# Autodesk Inventor assembly: TestAssembly_02
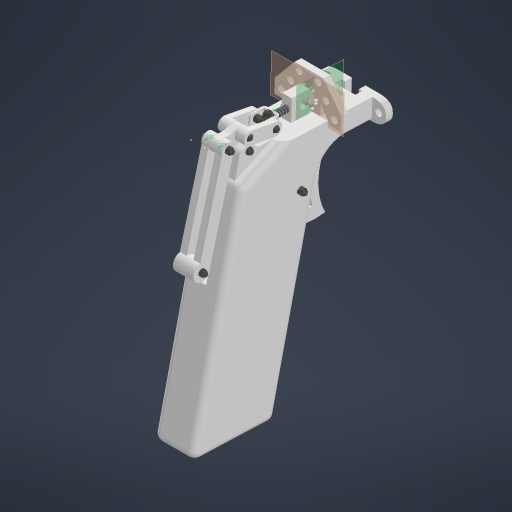
[picture p0: Inventor's stored thumbnail of the model, 512x512]
Saved by Autodesk Inventor 2024.1 (Build 281209000, 209)
## iProperties
Created: 2023-08-23
Part Number: TestAssembly_02
Document SubType Name: Assembly
Designer: Eleanor
Author: Eleanor
## Documents named in this file (13)
- C:\Users\Eleanor\Documents\Inventor\4.5mm ERS\TestAssembly_02.iam
- GripAssembly MK.001.iam
- C:\Users\Eleanor\Documents\Inventor\4.5mm ERS\Trigger.ipt
- C:\Users\Eleanor\Documents\Inventor\4.5mm ERS\TestAssembly_02\Design Accelerator\Clevis Pin Connection1.iam
- C:\Users\Eleanor\Documents\Inventor\4.5mm ERS\UpperLever.ipt
- C:\Users\Eleanor\Documents\Inventor\4.5mm ERS\LowerArm.ipt
- C:\Users\Eleanor\Documents\Inventor\4.5mm ERS\WireBarrelComponent_B.iam
- C:\Users\Eleanor\Documents\Inventor\Content Center Files\R2024\en-US\ISO 7380-1\ISO 7380-1 - M3 x 12.ipt
- C:\Users\Eleanor\Documents\Inventor\4.5mm ERS\FiringPinConnectorPlate.ipt
- C:\Users\Eleanor\Documents\Inventor\4.5mm ERS\FiringPinHolder.ipt
- C:\Users\Eleanor\Documents\Inventor\4.5mm ERS\Compress Spring12.ipt
- C:\Users\Eleanor\Documents\Inventor\4.5mm ERS\TestAssembly_02\Design Accelerator\Clevis Pin Connection2.iam
- C:\Users\Eleanor\Documents\Inventor\4.5mm ERS\Handgrip.iam
## Components (17 placed, 10 different names)
1. Trigger:1 — Mate:6, Mate:12, Mate:14, Mate:31, Mate:58, Mate:59, Mate:60
2. Clevis Pin Connection:1 [sub-assembly] — Mate:5, Mate:6, Mate:52, Mate:59, Mate:62
3. UpperLever:1 — Mate:13, Mate:15, Mate:19, Mate:21, Mate:54, Mate:61
4. LowerArm:1 — Mate:12, Mate:13, Mate:32, Mate:34, Mate:35, Mate:46, Mate:49
5. LowerArm:2 — Mate:14, Mate:15, Mate:57
6. WireBarrelComponent_B:1 [sub-assembly] — Mate:25, Mate:55, Mate:56
7. ISO 7380-1 M3 x 12:1 — Mate:25, Mate:26, Mate:29, Mate:30
8. FiringPinConnectorPlate:1 — Mate:19, Mate:20, Mate:23, Mate:28, Mate:37, Mate:38, Mate:40, Mate:44, Mate:50
9. FiringPinConnectorPlate:2 — Mate:21, Mate:28
10. FiringPinHolder:1 — Mate:20, Mate:23, Mate:26, Mate:29, Flush:2
11. Compress Spring1:1 — Mate:30, Flush:2
12. Clevis Pin Connection:2 [sub-assembly] — Mate:46, Mate:47, Mate:57
13. Clevis Pin Connection:3 [sub-assembly] — Mate:48, Mate:53, Mate:61
14. Clevis Pin Connection:4 [sub-assembly] — Mate:49
15. Clevis Pin Connection:5 [sub-assembly] — Mate:50
16. Clevis Pin Connection:6 [sub-assembly] — Mate:51
17. Handgrip:1 [sub-assembly] — Mate:52, Mate:53, Mate:54, Mate:55, Mate:56, Mate:58, Mate:60, Mate:62
## Relationships (47: Mate 46, Flush 1)
- Mate:3
- Mate:5: Clevis Pin Connection:1
- Mate:6: Trigger:1 ↔ Clevis Pin Connection:1
- Mate:12: Trigger:1 ↔ LowerArm:1
- Mate:13: UpperLever:1 ↔ LowerArm:1
- Mate:14: Trigger:1 ↔ LowerArm:2
- Mate:15: UpperLever:1 ↔ LowerArm:2
- Mate:19: UpperLever:1 ↔ FiringPinConnectorPlate:1
- Mate:20: FiringPinConnectorPlate:1 ↔ FiringPinHolder:1
- Mate:21: UpperLever:1 ↔ FiringPinConnectorPlate:2
- Mate:23: FiringPinConnectorPlate:1 ↔ FiringPinHolder:1
- Mate:25: WireBarrelComponent_B:1 ↔ ISO 7380-1 M3 x 12:1
- Mate:26: ISO 7380-1 M3 x 12:1 ↔ FiringPinHolder:1
- Mate:28: FiringPinConnectorPlate:1 ↔ FiringPinConnectorPlate:2
- Mate:29: ISO 7380-1 M3 x 12:1 ↔ FiringPinHolder:1
- Mate:30: ISO 7380-1 M3 x 12:1 ↔ Compress Spring1:1
- Flush:2: FiringPinHolder:1 ↔ Compress Spring1:1
- Mate:31: Trigger:1
- Mate:32: LowerArm:1
- Mate:33
- Mate:34: LowerArm:1
- Mate:35: LowerArm:1
- Mate:36
- Mate:37: FiringPinConnectorPlate:1
- Mate:38: FiringPinConnectorPlate:1
- Mate:39
- Mate:40: FiringPinConnectorPlate:1
- Mate:43
- Mate:44: FiringPinConnectorPlate:1
- Mate:45
- Mate:46: LowerArm:1 ↔ Clevis Pin Connection:2
- Mate:47: Clevis Pin Connection:2
- Mate:48: Clevis Pin Connection:3
- Mate:49: LowerArm:1 ↔ Clevis Pin Connection:4
- Mate:50: FiringPinConnectorPlate:1 ↔ Clevis Pin Connection:5
- Mate:51: Clevis Pin Connection:6
- Mate:52: Clevis Pin Connection:1 ↔ Handgrip:1
- Mate:53: Clevis Pin Connection:3 ↔ Handgrip:1
- Mate:54: UpperLever:1 ↔ Handgrip:1
- Mate:55: WireBarrelComponent_B:1 ↔ Handgrip:1
- Mate:56: WireBarrelComponent_B:1 ↔ Handgrip:1
- Mate:57: LowerArm:2 ↔ Clevis Pin Connection:2
- Mate:58: Trigger:1 ↔ Handgrip:1
- Mate:59: Trigger:1 ↔ Clevis Pin Connection:1
- Mate:60: Trigger:1 ↔ Handgrip:1
- Mate:61: UpperLever:1 ↔ Clevis Pin Connection:3
- Mate:62: Clevis Pin Connection:1 ↔ Handgrip:1
